# Autodesk Inventor assembly: ModuloLavaplatos
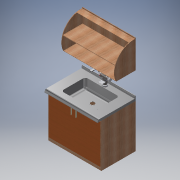
[picture p0: Inventor's stored thumbnail of the model, 180x180]
Saved by Autodesk Inventor 2016 (Build 200138000, 138)
## iProperties
Created: 2015-11-25
Part Number: ModuloLavaplatos
Document SubType Name: Assembly
Designer: Daniela
Author: Daniela
## Documents named in this file (6)
- D:\Documents\Carrera\11.Semeste_II_2015\Computacion_grafica\Proyecto\COCINA_FINAL\Cocina\ModuloLavaplatos_1.iam
- D:\Documents\Carrera\11.Semeste_II_2015\Computacion_grafica\Proyecto\COCINA_FINAL\Cocina\base_lavaplatos.ipt
- D:\Documents\Carrera\11.Semeste_II_2015\Computacion_grafica\Proyecto\COCINA_FINAL\Cocina\lavaplatos_1.ipt
- D:\Documents\Carrera\11.Semeste_II_2015\Computacion_grafica\Proyecto\COCINA_FINAL\Cocina\grifo.ipt
- D:\Documents\Carrera\11.Semeste_II_2015\Computacion_grafica\Proyecto\COCINA_FINAL\Cocina\puerta_lavaplatos.ipt
- D:\Documents\Carrera\11.Semeste_II_2015\Computacion_grafica\Proyecto\COCINA_FINAL\Cocina\manija.ipt
## Components (7 placed, 5 different names)
1. base_lavaplatos:1 — Mate:1, Flush:1, Flush:2, Mate:5, Mate:6, Mate:7
2. lavaplatos_1:1 — Mate:1, Flush:1, Flush:2, Mate:2, Mate:3
3. grifo:1 — Mate:2, Mate:3
4. puerta_lavaplatos:1 — Flush:3, Flush:4, Mate:4, Mate:9, Mate:11, Mate:12
5. puerta_lavaplatos:2 — Flush:3, Flush:4, Mate:4, Mate:5, Mate:6, Mate:7, Mate:8, Mate:10, Mate:13
6. manija:1 — Mate:8, Mate:10, Mate:13
7. manija:2 — Mate:9, Mate:11, Mate:12
## Relationships (17: Mate 13, Flush 4)
- Mate:1: base_lavaplatos:1 ↔ lavaplatos_1:1
- Flush:1: base_lavaplatos:1 ↔ lavaplatos_1:1
- Flush:2: base_lavaplatos:1 ↔ lavaplatos_1:1
- Mate:2: lavaplatos_1:1 ↔ grifo:1
- Mate:3: lavaplatos_1:1 ↔ grifo:1
- Flush:3: puerta_lavaplatos:1 ↔ puerta_lavaplatos:2
- Flush:4: puerta_lavaplatos:1 ↔ puerta_lavaplatos:2
- Mate:4: puerta_lavaplatos:1 ↔ puerta_lavaplatos:2
- Mate:5: base_lavaplatos:1 ↔ puerta_lavaplatos:2
- Mate:6 (-10 mm): base_lavaplatos:1 ↔ puerta_lavaplatos:2
- Mate:7 (-10 mm): base_lavaplatos:1 ↔ puerta_lavaplatos:2
- Mate:8: puerta_lavaplatos:2 ↔ manija:1
- Mate:9: puerta_lavaplatos:1 ↔ manija:2
- Mate:10: puerta_lavaplatos:2 ↔ manija:1
- Mate:11: puerta_lavaplatos:1 ↔ manija:2
- Mate:12: puerta_lavaplatos:1 ↔ manija:2
- Mate:13: puerta_lavaplatos:2 ↔ manija:1
